# Autodesk Inventor assembly: Motor
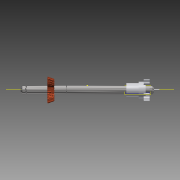
[picture p0: Inventor's stored thumbnail of the model, 180x180]
Saved by Autodesk Inventor 2015 (Build 190141000, 141)
## iProperties
Created: 2008-07-14
Part Number: Motor
Document SubType Name: Assembly
Designer: tangg
Mass: 130.161 g
Surface Area: 104.869 cm^2
Volume: 19.3028 cm^3
Density: 6.7431 g/cm^3
Author: tangg
## Documents named in this file (4)
- C:\Users\Aielloj\Downloads\inventor_2014_simulation\tutorial files\Dynamic Simulation 1 and 2\Motor.iam
- C:\Users\Aielloj\Downloads\inventor_2014_simulation\tutorial files\Dynamic Simulation 1 and 2\Motor shaft.ipt
- C:\Users\Aielloj\Downloads\inventor_2014_simulation\tutorial files\Dynamic Simulation 1 and 2\Cooling fan.ipt
- C:\Users\Aielloj\Downloads\inventor_2014_simulation\tutorial files\Dynamic Simulation 1 and 2\Bevel Gear11.ipt
## Components (3 placed, 3 different names)
1. Motor shaft:1 — Mate:1, Mate:2, Flush:1
2. Cooling fan:1 — Mate:1
3. Bevel Gear1:1 — Mate:2, Flush:1
## Relationships (3: Mate 2, Flush 1)
- Mate:1: Motor shaft:1 ↔ Cooling fan:1
- Mate:2: Motor shaft:1 ↔ Bevel Gear1:1
- Flush:1 (-30.56 mm): Motor shaft:1 ↔ Bevel Gear1:1
